# Autodesk Inventor assembly: new asembly
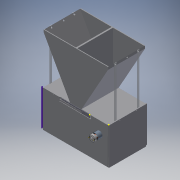
[picture p0: Inventor's stored thumbnail of the model, 180x180]
Saved by Autodesk Inventor 2019 (Build 230136000, 136)
## iProperties
Created: 2020-02-28
Part Number: new asembly
Document SubType Name: Assembly
Designer: KiranM
Author: KiranM
## Documents named in this file (10)
- C:\Users\KiranM\Desktop\Engineering_exploratiion\new asembly.iam
- C:\Users\KiranM\Desktop\Engineering_exploratiion\new container.ipt
- C:\Users\KiranM\Desktop\Engineering_exploratiion\new support.ipt
- C:\Users\KiranM\Desktop\Engineering_exploratiion\new Assembly2.iam
- C:\Users\KiranM\Desktop\Engineering_exploratiion\new  L clamp.ipt
- C:\Users\KiranM\Desktop\Engineering_exploratiion\back_motor 2.iam
- C:\Users\KiranM\Desktop\Engineering_exploratiion\new connect acr.ipt
- C:\Users\KiranM\Desktop\Engineering_exploratiion\new acr connect.ipt
- C:\Users\KiranM\Desktop\Engineering_exploratiion\new side wall.ipt
- C:\Users\KiranM\Desktop\Engineering_exploratiion\new lower.ipt
## Components (14 placed, 9 different names)
1. new container:1 — Mate:1, Mate:2, Mate:3, Mate:4, Mate:6, Mate:8, Mate:9, Mate:10, Mate:13, Mate:16
2. new support:1 — Mate:1
3. new support:2 — Mate:2
4. new support:3 — Mate:4
5. new support:4 — Mate:3
6. new Assembly2:1 [sub-assembly] — Mate:6, Mate:15
7. new  L clamp:2 — Mate:8
8. new  L clamp:3 — Mate:9
9. back_motor 2:1 [sub-assembly] — Mate:10, Mate:11, Mate:13
10. new connect acr:1 — Mate:11, Mate:14
11. new acr connect:1 — Mate:14, Mate:15
12. new side wall:1 — Mate:16
13. new lower:1
14. new side wall:2
## Relationships (13: Mate 13)
- Mate:1: new container:1 ↔ new support:1
- Mate:2: new container:1 ↔ new support:2
- Mate:3: new container:1 ↔ new support:4
- Mate:4: new container:1 ↔ new support:3
- Mate:6: new container:1 ↔ new Assembly2:1
- Mate:8: new container:1 ↔ new  L clamp:2
- Mate:9: new container:1 ↔ new  L clamp:3
- Mate:10: new container:1 ↔ back_motor 2:1
- Mate:11: back_motor 2:1 ↔ new connect acr:1
- Mate:13: new container:1 ↔ back_motor 2:1
- Mate:14: new connect acr:1 ↔ new acr connect:1
- Mate:15 (10 mm): new Assembly2:1 ↔ new acr connect:1
- Mate:16: new container:1 ↔ new side wall:1
